# Autodesk Inventor assembly: Mark 4.5
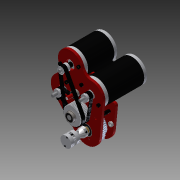
[picture p0: Inventor's stored thumbnail of the model, 180x180]
Saved by Autodesk Inventor 2013 (Build 170138000, 138)
## iProperties
Created: 2013-06-28
Part Number: Mark 4.5
Document SubType Name: Assembly
Designer: mvarma
Author: mvarma
## Documents named in this file (54)
- C:\Users\mvarma\Desktop\GRT 2013-2014 Gearbox\Mark 5\Mark 4.5.iam
- C:\Users\mvarma\Desktop\GRT 2013-2014 Gearbox\Mark 5\Plates\Mounting Plate.ipt
- C:\Users\mvarma\Desktop\GRT 2013-2014 Gearbox\Mark 5\Plates\Cim Plate.ipt
- C:\Users\mvarma\Desktop\GRT 2013-2014 Gearbox\Mark 5\Plates\Pnuematic Plate.ipt
- C:\Users\mvarma\Desktop\GRT 2013-2014 Gearbox\Mark 5\Plates\Main Connecting Standoff.ipt
- C:\Users\mvarma\Desktop\GRT 2013-2014 Gearbox\Mark 5\Pem Nuts\10-32 Clinch Style Pem Nut .091 Minimum Panel Thickness.ipt
- C:\Users\mvarma\Desktop\GRT 2013-2014 Gearbox\Mark 5\Pem Nuts\.25-20 Clinch Style Pem Nut .125 Minimum Panel Thickness.ipt
- C:\Users\mvarma\Desktop\GRT 2013-2014 Gearbox\Mark 5\Bearings\FR6-2ZZ - Hex.ipt
- C:\Users\mvarma\Desktop\GRT 2013-2014 Gearbox\Mark 5\Bearings\FR8-2RS.ipt
- C:\Users\mvarma\Desktop\GRT 2013-2014 Gearbox\Mark 5\Bearings\FR6-2RS.ipt
- C:\Users\mvarma\Desktop\GRT 2013-2014 Gearbox\Mark 5\Encoder\Encoder Mount.ipt
- C:\Users\mvarma\Desktop\GRT 2013-2014 Gearbox\Mark 5\Encoder\S4-120-250-N-S-B.ipt
- C:\Users\mvarma\Desktop\GRT 2013-2014 Gearbox\Mark 5\Shafts\Cluster Shaft.ipt
- C:\Users\mvarma\Desktop\GRT 2013-2014 Gearbox\Mark 5\Shafts\Flexible Shaft Coupler 6208K411.ipt
- C:\Users\mvarma\Desktop\GRT 2013-2014 Gearbox\Mark 5\Spacers\Cluster Shaft Spacer.ipt
- C:\Users\mvarma\Desktop\GRT 2013-2014 Gearbox\Mark 5\Gears\15T 20DP - .375 Hex Bore.ipt
- C:\Users\mvarma\Desktop\GRT 2013-2014 Gearbox\Mark 5\Gears\28T 20DP - .375 Hex Bore.ipt
- C:\Users\mvarma\Desktop\GRT 2013-2014 Gearbox\Mark 5\Shafts\Output Shaft.ipt
- C:\Users\mvarma\Desktop\GRT 2013-2014 Gearbox\Mark 5\Spacers\Shim 10 thou .500 Bore.ipt
- C:\Users\mvarma\Desktop\GRT 2013-2014 Gearbox\Mark 5\Bearings\R10-Open.ipt
- C:\Users\mvarma\Desktop\GRT 2013-2014 Gearbox\Mark 5\Gears\35T 20DP - .188 Ball Shifting Bore.ipt
- C:\Users\mvarma\Desktop\GRT 2013-2014 Gearbox\Mark 5\Gears\48T 20DP - .188 Ball Shifting Bore.ipt
- C:\Users\mvarma\Desktop\GRT 2013-2014 Gearbox\Mark 5\Bearings\Thrust Bearing Washer - .6250 Bore.ipt
- C:\Users\mvarma\Desktop\GRT 2013-2014 Gearbox\Mark 5\Spacers\Shim 10 thou .625 Bore.ipt
- C:\Users\mvarma\Desktop\GRT 2013-2014 Gearbox\Mark 5\Spacers\Shim 10 thou .375 Bore.ipt
- C:\Users\mvarma\Desktop\GRT 2013-2014 Gearbox\Mark 5\Pulleys\48T 3mm GT2 - .375 Hex Broach - Hubless.ipt
- C:\Users\mvarma\Desktop\GRT 2013-2014 Gearbox\Mark 5\Pem Nuts\4-40 Clinch Style Pem Nut .091 Minimum Panel Thickness.ipt
- C:\Users\mvarma\Desktop\GRT 2013-2014 Gearbox\Mark 5\Shafts\Tensioning Shaft.ipt
- C:\Users\mvarma\Desktop\GRT 2013-2014 Gearbox\Mark 5\Spacers\Belt Shaft Spacer 2.ipt
- C:\Users\mvarma\Desktop\GRT 2013-2014 Gearbox\Mark 5\Bearings\R4-2RS.ipt
- C:\Users\mvarma\Desktop\GRT 2013-2014 Gearbox\Mark 5\Motors\CIM Can.ipt
- C:\Users\mvarma\Desktop\GRT 2013-2014 Gearbox\Mark 5\Motors\Mini CIM Can.ipt
- C:\Users\mvarma\Desktop\GRT 2013-2014 Gearbox\Mark 5\Motors\Rotor.ipt
- C:\Users\mvarma\Desktop\GRT 2013-2014 Gearbox\Mark 5\Belts\267 mm Belt.ipt
- C:\Users\mvarma\Desktop\GRT 2013-2014 Gearbox\Mark 5\Belts\285 mm Belt.ipt
- C:\Users\mvarma\Desktop\GRT 2013-2014 Gearbox\Mark 5\Pulleys\16T 3mm GT2 - 8mm Key Broach.ipt
- C:\Users\mvarma\Desktop\GRT 2013-2014 Gearbox\Mark 5\Spacers\Cim Spacer.ipt
- C:\Users\mvarma\Desktop\GRT 2013-2014 Gearbox\Mark 5\Spacers\MiniCim Spacer.ipt
- C:\Users\mvarma\Desktop\GRT 2013-2014 Gearbox\Mark 5\Shafts\Ball Shifting Shaft.ipt
- C:\Users\mvarma\Desktop\GRT 2013-2014 Gearbox\Mark 5\Shafts\Output Shaft Insert.ipt
- C:\Users\mvarma\Desktop\GRT 2013-2014 Gearbox\Mark 5\Bearings\R3-2RS.ipt
- C:\Users\mvarma\Desktop\GRT 2013-2014 Gearbox\Mark 5\.0625 Spring Pin .2500 Long.ipt
- C:\Users\mvarma\Desktop\GRT 2013-2014 Gearbox\Mark 5\Pneumatic\Pneumatic Connector -Actuator Side.ipt
- C:\Users\mvarma\Desktop\GRT 2013-2014 Gearbox\Mark 5\Pneumatic\Pneumatic Connector -Shaft Side Cover.ipt
- C:\Users\mvarma\Desktop\GRT 2013-2014 Gearbox\Mark 5\Pneumatic\Pancake Pneumatic.iam
- C:\Users\mvarma\Desktop\GRT 2013-2014 Gearbox\Mark 5\Bolts\Button Head Cap Screw 4-40 Thread .125 Length.ipt
- C:\Users\mvarma\Desktop\GRT 2013-2014 Gearbox\Mark 5\Shafts\Output Shaft Hex Sleave.ipt
- C:\Users\mvarma\Desktop\GRT 2013-2014 Gearbox\Mark 5\Frame Segment.ipt
- C:\Users\mvarma\Desktop\GRT 2013-2014 Gearbox\Mark 5\Bolts\Socket Head Cap Screw 6-32 Thread 1.000 Length.ipt
- C:\Users\mvarma\Desktop\GRT 2013-2014 Gearbox\Mark 5\Plates\Cim Adjustment Block.ipt
- C:\Users\mvarma\Desktop\GRT 2013-2014 Gearbox\Mark 5\Bolts\Socket Head Cap Screw 6-32 Thread .500 Length.ipt
- C:\Users\mvarma\Desktop\GRT 2013-2014 Gearbox\Mark 5\Bolts\Socket Head Cap Screw 6-32 Thread .375 Length.ipt
- C:\Users\mvarma\Desktop\GRT 2013-2014 Gearbox\Mark 5\Bolts\Socket Head Cap Screw 10-32 Thread .750 Length.ipt
- C:\Users\mvarma\Desktop\GRT 2013-2014 Gearbox\Mark 5\Bolts\Socket Head Cap Screw 4-40 Thread 1.000 Length.ipt
## Components (85 placed, 53 different names)
1. Frame Segment:1 — Mate:228, Mate:229
2. Socket Head Cap Screw 4-40 Thread 1.000 Length:1 — Mate:270, Mate:272
3. Socket Head Cap Screw 4-40 Thread 1.000 Length:2 — Mate:271, Mate:273
4. 267 mm Belt:1 — Mate:174, Mate:175, Mate:179, Flush:2, Flush:3
5. 285 mm Belt:1 — Mate:176, Mate:177, Mate:178, Flush:1
6. Socket Head Cap Screw 6-32 Thread 1.000 Length:1 — Mate:232, Mate:234
7. Socket Head Cap Screw 6-32 Thread 1.000 Length:2 — Mate:231, Mate:233
8. S4-120-250-N-S-B:1 — Mate:66, Mate:67
9. Flexible Shaft Coupler 6208K411:1 — Mate:64, Mate:65, Mate:66, Mate:67
10. Encoder Mount:1 — Mate:225, Mate:226, Mate:227, Mate:231, Mate:232, Mate:233, Mate:234
11. Cim Spacer:1 — Mate:184, Mate:185
12. MiniCim Spacer:1 — Mate:187, Mate:188
13. Cim Spacer:2 — Mate:183, Mate:186
14. CIM Can:1 — Mate:153, Mate:154, Mate:155, Mate:163, Mate:166, Mate:185
15. CIM Can:2 — Mate:156, Mate:157, Mate:158, Mate:164, Mate:165, Mate:186
16. Mini CIM Can:1 — Mate:159, Mate:160, Mate:161, Mate:162, Mate:167, Mate:188, Mate:254
17. Rotor:1 — Mate:164, Mate:165, Mate:175, Mate:181, Mate:183
18. Rotor:2 — Mate:163, Mate:166, Mate:180, Mate:184
19. Rotor:3 — Mate:162, Mate:167, Mate:177, Mate:182, Mate:187
20. Pneumatic Connector -Actuator Side:1 — Mate:196, Mate:197, Mate:198, Mate:203, Mate:210, Mate:211
21. Pneumatic Connector -Shaft Side Cover:1 — Mate:196, Mate:197, Mate:198, Mate:201, Mate:214, Mate:219, Mate:220, Mate:221, Mate:222
22. Pancake Pneumatic:1 [sub-assembly] — Mate:209, Mate:210, Mate:211, Mate:212, Mate:213, Mate:270, Mate:271, Mate:272, Mate:273
23. Button Head Cap Screw 4-40 Thread .125 Length:1 — Mate:221, Mate:222
24. Button Head Cap Screw 4-40 Thread .125 Length:2 — Mate:219, Mate:220
25. 16T 3mm GT2 - 8mm Key Broach:1 — Mate:180, Flush:3
26. 16T 3mm GT2 - 8mm Key Broach:2 — Mate:181, Flush:2
27. 16T 3mm GT2 - 8mm Key Broach:3 — Mate:182, Flush:1
28. Main Connecting Standoff:3 — Mate:3, Mate:12, Mate:27, Mate:140
29. Main Connecting Standoff:5 — Mate:5, Mate:16, Mate:25
30. Main Connecting Standoff:8 — Mate:8, Mate:19, Mate:24
31. Socket Head Cap Screw 10-32 Thread .750 Length:1 — Mate:262, Mate:263
32. Socket Head Cap Screw 10-32 Thread .750 Length:2 — Mate:252, Mate:253
33. Socket Head Cap Screw 10-32 Thread .750 Length:3 — Mate:254, Mate:255
34. Socket Head Cap Screw 10-32 Thread .750 Length:4 — Mate:260, Mate:261
35. Socket Head Cap Screw 10-32 Thread .750 Length:5 — Mate:256, Mate:259
36. Socket Head Cap Screw 10-32 Thread .750 Length:6 — Mate:257, Mate:258
37. Mounting Plate:1 — Mate:3, Mate:5, Mate:8, Mate:24, Mate:25, Mate:27, Mate:31, Mate:34, Mate:36, Mate:40, Mate:42, Mate:45, Mate:48, Mate:49, Mate:50, Mate:51, Mate:53, Mate:55, Mate:56, Mate:57, Mate:68, Mate:73, Mate:74, Mate:225, Mate:226, Mate:227, Mate:229, Mate:235, Mate:236, Mate:237, Mate:243, Mate:244, Mate:245
38. FR8-2RS:1 — Mate:53, Mate:55, Mate:80, Mate:83
39. FR6-2RS:1 — Mate:56, Mate:57, Mate:72
40. Cim Plate:1 — Mate:12, Mate:16, Mate:19, Mate:58, Mate:59, Mate:60, Mate:61, Mate:114, Mate:115, Mate:139, Mate:140, Mate:141, Mate:142, Mate:153, Mate:154, Mate:155, Mate:156, Mate:157, Mate:158, Mate:159, Mate:160, Mate:161, Mate:174, Mate:176, Mate:252, Mate:253, Mate:255, Mate:256, Mate:257, Mate:258, Mate:259, Mate:260, Mate:261, Mate:262, Mate:263
41. FR6-2ZZ - Hex:1 — Mate:60, Mate:61, Mate:79, Mate:125
42. FR8-2RS:2 — Mate:58, Mate:59, Mate:214
43. Pnuematic Plate:1 — Mate:114, Mate:115, Mate:133, Mate:134, Mate:139, Mate:146, Mate:209, Mate:212, Mate:213, Mate:215, Mate:216, Mate:217, Mate:218
44. FR6-2RS:2 — Mate:133, Mate:134
45. Ball Shifting Shaft:1 — Mate:191, Mate:192, Mate:193, Mate:194, Mate:195, Mate:201
46. R3-2RS:1 — Mate:192, Mate:193, Mate:203
47. .0625 Spring Pin .2500 Long:1 — Mate:194, Mate:195
48. Cluster Shaft:1 — Mate:64, Mate:65, Mate:68, Mate:71, Mate:75, Mate:76, Mate:79, Mate:123, Mate:124, Mate:126, Mate:127, Mate:128, Mate:129
49. Cluster Shaft Spacer:1 — Mate:71, Mate:72, Mate:78
50. 15T 20DP - .375 Hex Bore:1 — Mate:74, Mate:76, Mate:77
51. 28T 20DP - .375 Hex Bore:1 — Mate:73, Mate:75, Mate:77, Mate:78
52. Shim 10 thou .375 Bore:1 — Mate:123, Mate:132
53. Shim 10 thou .500 Bore:2 — Mate:124, Mate:125, Mate:131
54. 48T 3mm GT2 - .375 Hex Broach - Hubless:1 — Mate:126, Mate:128, Mate:130, Mate:132, Mate:178
55. 48T 3mm GT2 - .375 Hex Broach - Hubless:2 — Mate:127, Mate:129, Mate:130, Mate:131, Mate:179
56. Output Shaft Insert:1 — Mate:189, Mate:190, Mate:191
57. Shim 10 thou .625 Bore:1 — Mate:96, Mate:97
58. Thrust Bearing Washer - .6250 Bore:2 — Mate:94, Mate:95, Mate:97
59. 48T 20DP - .188 Ball Shifting Bore:1 — Mate:92, Mate:93, Mate:95
60. R10-Open:1 — Mate:90, Mate:91, Mate:93
61. Thrust Bearing Washer - .6250 Bore:1 — Mate:88, Mate:89, Mate:91
62. 35T 20DP - .188 Ball Shifting Bore:1 — Mate:86, Mate:87, Mate:89
63. R10-Open:2 — Mate:84, Mate:85, Mate:87
64. Shim 10 thou .500 Bore:1 — Mate:81, Mate:82, Mate:83, Mate:85
65. Output Shaft:1 — Mate:80, Mate:81, Mate:82, Mate:84, Mate:86, Mate:88, Mate:90, Mate:92, Mate:94, Mate:96, Mate:189, Mate:190, Mate:223, Mate:224, Flush:4, Mate:228
66. Output Shaft Hex Sleave:1 — Mate:223, Mate:224, Flush:4
67. Tensioning Shaft:1 — Mate:141, Mate:142, Mate:143, Mate:149
68. Belt Shaft Spacer 2:1 — Mate:143, Mate:146, Mate:150
69. R4-2RS:1 — Mate:147, Mate:148, Mate:149, Mate:150
70. R4-2RS:2 — Mate:147, Mate:148
71. Cim Adjustment Block:1 — Mate:235, Mate:236, Mate:237, Mate:238, Mate:239, Mate:240, Mate:241, Mate:251
72. Cim Adjustment Block:2 — Mate:243, Mate:244, Mate:245, Mate:246, Mate:247, Mate:248, Mate:249, Mate:250
73. Socket Head Cap Screw 6-32 Thread .500 Length:1 — Mate:239, Mate:240
74. Socket Head Cap Screw 6-32 Thread .500 Length:2 — Mate:238, Mate:241
75. Socket Head Cap Screw 6-32 Thread .375 Length:2 — Mate:251
76. Socket Head Cap Screw 6-32 Thread .500 Length:4 — Mate:246, Mate:249
77. Socket Head Cap Screw 6-32 Thread .500 Length:5 — Mate:247, Mate:248
78. Socket Head Cap Screw 6-32 Thread .375 Length:1 — Mate:250
79. 10-32 Clinch Style Pem Nut .091 Minimum Panel Thickness:2 — Mate:34, Mate:40
80. 10-32 Clinch Style Pem Nut .091 Minimum Panel Thickness:4 — Mate:31, Mate:42
81. 10-32 Clinch Style Pem Nut .091 Minimum Panel Thickness:8 — Mate:36, Mate:45
82. .25-20 Clinch Style Pem Nut .125 Minimum Panel Thickness:1 — Mate:49, Mate:50
83. .25-20 Clinch Style Pem Nut .125 Minimum Panel Thickness:2 — Mate:48, Mate:51
84. 4-40 Clinch Style Pem Nut .091 Minimum Panel Thickness:1 — Mate:216, Mate:218
85. 4-40 Clinch Style Pem Nut .091 Minimum Panel Thickness:2 — Mate:215, Mate:217
## Relationships (188: Mate 182, Flush 4, Tangent 2)
- Mate:3: Main Connecting Standoff:3 ↔ Mounting Plate:1
- Mate:5: Main Connecting Standoff:5 ↔ Mounting Plate:1
- Mate:8: Main Connecting Standoff:8 ↔ Mounting Plate:1
- Mate:12: Main Connecting Standoff:3 ↔ Cim Plate:1
- Mate:16: Main Connecting Standoff:5 ↔ Cim Plate:1
- Mate:19: Main Connecting Standoff:8 ↔ Cim Plate:1
- Mate:24: Main Connecting Standoff:8 ↔ Mounting Plate:1
- Mate:25: Main Connecting Standoff:5 ↔ Mounting Plate:1
- Mate:27: Main Connecting Standoff:3 ↔ Mounting Plate:1
- Mate:31: Mounting Plate:1 ↔ 10-32 Clinch Style Pem Nut .091 Minimum Panel Thickness:4
- Mate:34: Mounting Plate:1 ↔ 10-32 Clinch Style Pem Nut .091 Minimum Panel Thickness:2
- Mate:36: Mounting Plate:1 ↔ 10-32 Clinch Style Pem Nut .091 Minimum Panel Thickness:8
- Mate:40: Mounting Plate:1 ↔ 10-32 Clinch Style Pem Nut .091 Minimum Panel Thickness:2
- Mate:42: Mounting Plate:1 ↔ 10-32 Clinch Style Pem Nut .091 Minimum Panel Thickness:4
- Mate:45: Mounting Plate:1 ↔ 10-32 Clinch Style Pem Nut .091 Minimum Panel Thickness:8
- Mate:48: Mounting Plate:1 ↔ .25-20 Clinch Style Pem Nut .125 Minimum Panel Thickness:2
- Mate:49: Mounting Plate:1 ↔ .25-20 Clinch Style Pem Nut .125 Minimum Panel Thickness:1
- Mate:50: Mounting Plate:1 ↔ .25-20 Clinch Style Pem Nut .125 Minimum Panel Thickness:1
- Mate:51: Mounting Plate:1 ↔ .25-20 Clinch Style Pem Nut .125 Minimum Panel Thickness:2
- Mate:53: Mounting Plate:1 ↔ FR8-2RS:1
- Mate:55: Mounting Plate:1 ↔ FR8-2RS:1
- Mate:56: Mounting Plate:1 ↔ FR6-2RS:1
- Mate:57: Mounting Plate:1 ↔ FR6-2RS:1
- Mate:58: Cim Plate:1 ↔ FR8-2RS:2
- Mate:59: Cim Plate:1 ↔ FR8-2RS:2
- Mate:60: Cim Plate:1 ↔ FR6-2ZZ - Hex:1
- Mate:61: Cim Plate:1 ↔ FR6-2ZZ - Hex:1
- Mate:64: Flexible Shaft Coupler 6208K411:1 ↔ Cluster Shaft:1
- Mate:65: Flexible Shaft Coupler 6208K411:1 ↔ Cluster Shaft:1
- Mate:66: S4-120-250-N-S-B:1 ↔ Flexible Shaft Coupler 6208K411:1
- Mate:67: S4-120-250-N-S-B:1 ↔ Flexible Shaft Coupler 6208K411:1
- Mate:68: Mounting Plate:1 ↔ Cluster Shaft:1
- Mate:71: Cluster Shaft:1 ↔ Cluster Shaft Spacer:1
- Mate:72: FR6-2RS:1 ↔ Cluster Shaft Spacer:1
- Mate:73: Mounting Plate:1 ↔ 28T 20DP - .375 Hex Bore:1
- Mate:74: Mounting Plate:1 ↔ 15T 20DP - .375 Hex Bore:1
- Mate:75: Cluster Shaft:1 ↔ 28T 20DP - .375 Hex Bore:1
- Mate:76: Cluster Shaft:1 ↔ 15T 20DP - .375 Hex Bore:1
- Mate:77: 15T 20DP - .375 Hex Bore:1 ↔ 28T 20DP - .375 Hex Bore:1
- Mate:78: Cluster Shaft Spacer:1 ↔ 28T 20DP - .375 Hex Bore:1
- Mate:79: FR6-2ZZ - Hex:1 ↔ Cluster Shaft:1
- Mate:80: FR8-2RS:1 ↔ Output Shaft:1
- Mate:81: Shim 10 thou .500 Bore:1 ↔ Output Shaft:1
- Mate:82: Shim 10 thou .500 Bore:1 ↔ Output Shaft:1
- Mate:83: FR8-2RS:1 ↔ Shim 10 thou .500 Bore:1
- Mate:84: R10-Open:2 ↔ Output Shaft:1
- Mate:85: R10-Open:2 ↔ Shim 10 thou .500 Bore:1
- Mate:86: 35T 20DP - .188 Ball Shifting Bore:1 ↔ Output Shaft:1
- Mate:87: 35T 20DP - .188 Ball Shifting Bore:1 ↔ R10-Open:2
- Mate:88: Thrust Bearing Washer - .6250 Bore:1 ↔ Output Shaft:1
- Mate:89: Thrust Bearing Washer - .6250 Bore:1 ↔ 35T 20DP - .188 Ball Shifting Bore:1
- Mate:90: R10-Open:1 ↔ Output Shaft:1
- Mate:91: R10-Open:1 ↔ Thrust Bearing Washer - .6250 Bore:1
- Mate:92: 48T 20DP - .188 Ball Shifting Bore:1 ↔ Output Shaft:1
- Mate:93: 48T 20DP - .188 Ball Shifting Bore:1 ↔ R10-Open:1
- Mate:94: Thrust Bearing Washer - .6250 Bore:2 ↔ Output Shaft:1
- Mate:95: Thrust Bearing Washer - .6250 Bore:2 ↔ 48T 20DP - .188 Ball Shifting Bore:1
- Mate:96: Shim 10 thou .625 Bore:1 ↔ Output Shaft:1
- Mate:97: Shim 10 thou .625 Bore:1 ↔ Thrust Bearing Washer - .6250 Bore:2
- Mate:114: Cim Plate:1 ↔ Pnuematic Plate:1
- Mate:115: Cim Plate:1 ↔ Pnuematic Plate:1
- Mate:123: Cluster Shaft:1 ↔ Shim 10 thou .375 Bore:1
- Mate:124: Cluster Shaft:1 ↔ Shim 10 thou .500 Bore:2
- Mate:125: FR6-2ZZ - Hex:1 ↔ Shim 10 thou .500 Bore:2
- Mate:126: Cluster Shaft:1 ↔ 48T 3mm GT2 - .375 Hex Broach - Hubless:1
- Mate:127: Cluster Shaft:1 ↔ 48T 3mm GT2 - .375 Hex Broach - Hubless:2
- Mate:128: Cluster Shaft:1 ↔ 48T 3mm GT2 - .375 Hex Broach - Hubless:1
- Mate:129: Cluster Shaft:1 ↔ 48T 3mm GT2 - .375 Hex Broach - Hubless:2
- Mate:130: 48T 3mm GT2 - .375 Hex Broach - Hubless:1 ↔ 48T 3mm GT2 - .375 Hex Broach - Hubless:2
- Mate:131: Shim 10 thou .500 Bore:2 ↔ 48T 3mm GT2 - .375 Hex Broach - Hubless:2
- Mate:132: Shim 10 thou .375 Bore:1 ↔ 48T 3mm GT2 - .375 Hex Broach - Hubless:1
- Mate:133: Pnuematic Plate:1 ↔ FR6-2RS:2
- Mate:134: Pnuematic Plate:1 ↔ FR6-2RS:2
- Mate:139: Cim Plate:1 ↔ Pnuematic Plate:1
- Mate:140: Main Connecting Standoff:3 ↔ Cim Plate:1
- Mate:141: Cim Plate:1 ↔ Tensioning Shaft:1
- Mate:142: Cim Plate:1 ↔ Tensioning Shaft:1
- Mate:143: Tensioning Shaft:1 ↔ Belt Shaft Spacer 2:1
- Mate:146: Pnuematic Plate:1 ↔ Belt Shaft Spacer 2:1
- Mate:147: R4-2RS:1 ↔ R4-2RS:2
- Mate:148: R4-2RS:1 ↔ R4-2RS:2
- Mate:149: Tensioning Shaft:1 ↔ R4-2RS:1
- Mate:150: Belt Shaft Spacer 2:1 ↔ R4-2RS:1
- Mate:153: CIM Can:1 ↔ Cim Plate:1
- Mate:154: CIM Can:1 ↔ Cim Plate:1
- Mate:155: CIM Can:1 ↔ Cim Plate:1
- Mate:156: CIM Can:2 ↔ Cim Plate:1
- Mate:157: CIM Can:2 ↔ Cim Plate:1
- Mate:158: CIM Can:2 ↔ Cim Plate:1
- Mate:159: Mini CIM Can:1 ↔ Cim Plate:1
- Mate:160: Mini CIM Can:1 ↔ Cim Plate:1
- Mate:161: Mini CIM Can:1 ↔ Cim Plate:1
- Mate:162: Mini CIM Can:1 ↔ Rotor:3
- Mate:163: CIM Can:1 ↔ Rotor:2
- Mate:164: CIM Can:2 ↔ Rotor:1
- Mate:165: CIM Can:2 ↔ Rotor:1
- Mate:166: CIM Can:1 ↔ Rotor:2
- Mate:167: Mini CIM Can:1 ↔ Rotor:3
- Mate:174: 267 mm Belt:1 ↔ Cim Plate:1
- Mate:175: 267 mm Belt:1 ↔ Rotor:1
- Mate:176: 285 mm Belt:1 ↔ Cim Plate:1
- Mate:177: 285 mm Belt:1 ↔ Rotor:3
- Mate:178: 285 mm Belt:1 ↔ 48T 3mm GT2 - .375 Hex Broach - Hubless:1
- Mate:179: 267 mm Belt:1 ↔ 48T 3mm GT2 - .375 Hex Broach - Hubless:2
- Mate:180: Rotor:2 ↔ 16T 3mm GT2 - 8mm Key Broach:1
- Mate:181: Rotor:1 ↔ 16T 3mm GT2 - 8mm Key Broach:2
- Mate:182: Rotor:3 ↔ 16T 3mm GT2 - 8mm Key Broach:3
- Flush:1: 285 mm Belt:1 ↔ 16T 3mm GT2 - 8mm Key Broach:3
- Flush:2: 267 mm Belt:1 ↔ 16T 3mm GT2 - 8mm Key Broach:2
- Flush:3: 267 mm Belt:1 ↔ 16T 3mm GT2 - 8mm Key Broach:1
- Mate:183: Cim Spacer:2 ↔ Rotor:1
- Mate:184: Cim Spacer:1 ↔ Rotor:2
- Mate:185: Cim Spacer:1 ↔ CIM Can:1
- Mate:186: Cim Spacer:2 ↔ CIM Can:2
- Mate:187: MiniCim Spacer:1 ↔ Rotor:3
- Mate:188: MiniCim Spacer:1 ↔ Mini CIM Can:1
- Mate:189: Output Shaft Insert:1 ↔ Output Shaft:1
- Mate:190: Output Shaft Insert:1 ↔ Output Shaft:1
- Mate:191: Ball Shifting Shaft:1 ↔ Output Shaft Insert:1
- Mate:192: Ball Shifting Shaft:1 ↔ R3-2RS:1
- Mate:193: Ball Shifting Shaft:1 ↔ R3-2RS:1
- Mate:194: Ball Shifting Shaft:1 ↔ .0625 Spring Pin .2500 Long:1
- Mate:195: Ball Shifting Shaft:1 ↔ .0625 Spring Pin .2500 Long:1
- Mate:196: Pneumatic Connector -Actuator Side:1 ↔ Pneumatic Connector -Shaft Side Cover:1
- Mate:197: Pneumatic Connector -Actuator Side:1 ↔ Pneumatic Connector -Shaft Side Cover:1
- Mate:198: Pneumatic Connector -Actuator Side:1 ↔ Pneumatic Connector -Shaft Side Cover:1
- Mate:201: Pneumatic Connector -Shaft Side Cover:1 ↔ Ball Shifting Shaft:1
- Mate:203: Pneumatic Connector -Actuator Side:1 ↔ R3-2RS:1
- Mate:209: Pancake Pneumatic:1 ↔ Pnuematic Plate:1
- Mate:210: Pneumatic Connector -Actuator Side:1 ↔ Pancake Pneumatic:1
- Mate:211: Pneumatic Connector -Actuator Side:1 ↔ Pancake Pneumatic:1
- Mate:212: Pancake Pneumatic:1 ↔ Pnuematic Plate:1
- Mate:213: Pancake Pneumatic:1 ↔ Pnuematic Plate:1
- Mate:214 (8.8582 mm): Pneumatic Connector -Shaft Side Cover:1 ↔ FR8-2RS:2
- Mate:215: Pnuematic Plate:1 ↔ 4-40 Clinch Style Pem Nut .091 Minimum Panel Thickness:2
- Mate:216: Pnuematic Plate:1 ↔ 4-40 Clinch Style Pem Nut .091 Minimum Panel Thickness:1
- Mate:217: Pnuematic Plate:1 ↔ 4-40 Clinch Style Pem Nut .091 Minimum Panel Thickness:2
- Mate:218: Pnuematic Plate:1 ↔ 4-40 Clinch Style Pem Nut .091 Minimum Panel Thickness:1
- Mate:219: Pneumatic Connector -Shaft Side Cover:1 ↔ Button Head Cap Screw 4-40 Thread .125 Length:2
- Mate:220: Pneumatic Connector -Shaft Side Cover:1 ↔ Button Head Cap Screw 4-40 Thread .125 Length:2
- Mate:221: Pneumatic Connector -Shaft Side Cover:1 ↔ Button Head Cap Screw 4-40 Thread .125 Length:1
- Mate:222: Pneumatic Connector -Shaft Side Cover:1 ↔ Button Head Cap Screw 4-40 Thread .125 Length:1
- Mate:223: Output Shaft:1 ↔ Output Shaft Hex Sleave:1
- Mate:224: Output Shaft:1 ↔ Output Shaft Hex Sleave:1
- Flush:4: Output Shaft:1 ↔ Output Shaft Hex Sleave:1
- Mate:225: Encoder Mount:1 ↔ Mounting Plate:1
- Mate:226: Encoder Mount:1 ↔ Mounting Plate:1
- Mate:227: Encoder Mount:1 ↔ Mounting Plate:1
- Mate:228: Frame Segment:1 ↔ Output Shaft:1
- Mate:229: Frame Segment:1 ↔ Mounting Plate:1
- Mate:231: Socket Head Cap Screw 6-32 Thread 1.000 Length:2 ↔ Encoder Mount:1
- Mate:232: Socket Head Cap Screw 6-32 Thread 1.000 Length:1 ↔ Encoder Mount:1
- Mate:233: Socket Head Cap Screw 6-32 Thread 1.000 Length:2 ↔ Encoder Mount:1
- Mate:234: Socket Head Cap Screw 6-32 Thread 1.000 Length:1 ↔ Encoder Mount:1
- Mate:235: Mounting Plate:1 ↔ Cim Adjustment Block:1
- Mate:236: Mounting Plate:1 ↔ Cim Adjustment Block:1
- Mate:237: Mounting Plate:1 ↔ Cim Adjustment Block:1
- Mate:238: Cim Adjustment Block:1 ↔ Socket Head Cap Screw 6-32 Thread .500 Length:2
- Mate:239: Cim Adjustment Block:1 ↔ Socket Head Cap Screw 6-32 Thread .500 Length:1
- Mate:240: Cim Adjustment Block:1 ↔ Socket Head Cap Screw 6-32 Thread .500 Length:1
- Mate:241: Cim Adjustment Block:1 ↔ Socket Head Cap Screw 6-32 Thread .500 Length:2
- [Tangent]: CIM Can:2 ↔ Socket Head Cap Screw 6-32 Thread .375 Length:2
- Mate:243: Mounting Plate:1 ↔ Cim Adjustment Block:2
- Mate:244: Mounting Plate:1 ↔ Cim Adjustment Block:2
- Mate:245: Mounting Plate:1 ↔ Cim Adjustment Block:2
- Mate:246: Cim Adjustment Block:2 ↔ Socket Head Cap Screw 6-32 Thread .500 Length:4
- Mate:247: Cim Adjustment Block:2 ↔ Socket Head Cap Screw 6-32 Thread .500 Length:5
- Mate:248: Cim Adjustment Block:2 ↔ Socket Head Cap Screw 6-32 Thread .500 Length:5
- Mate:249: Cim Adjustment Block:2 ↔ Socket Head Cap Screw 6-32 Thread .500 Length:4
- [Tangent]: Mini CIM Can:1 ↔ Socket Head Cap Screw 6-32 Thread .375 Length:1
- Mate:250: Cim Adjustment Block:2 ↔ Socket Head Cap Screw 6-32 Thread .375 Length:1
- Mate:251: Cim Adjustment Block:1 ↔ Socket Head Cap Screw 6-32 Thread .375 Length:2
- Mate:252: Socket Head Cap Screw 10-32 Thread .750 Length:2 ↔ Cim Plate:1
- Mate:253: Socket Head Cap Screw 10-32 Thread .750 Length:2 ↔ Cim Plate:1
- Mate:254: Mini CIM Can:1 ↔ Socket Head Cap Screw 10-32 Thread .750 Length:3
- Mate:255: Socket Head Cap Screw 10-32 Thread .750 Length:3 ↔ Cim Plate:1
- Mate:256: Socket Head Cap Screw 10-32 Thread .750 Length:5 ↔ Cim Plate:1
- Mate:257: Socket Head Cap Screw 10-32 Thread .750 Length:6 ↔ Cim Plate:1
- Mate:258: Socket Head Cap Screw 10-32 Thread .750 Length:6 ↔ Cim Plate:1
- Mate:259: Socket Head Cap Screw 10-32 Thread .750 Length:5 ↔ Cim Plate:1
- Mate:260: Socket Head Cap Screw 10-32 Thread .750 Length:4 ↔ Cim Plate:1
- Mate:261: Socket Head Cap Screw 10-32 Thread .750 Length:4 ↔ Cim Plate:1
- Mate:262: Socket Head Cap Screw 10-32 Thread .750 Length:1 ↔ Cim Plate:1
- Mate:263: Socket Head Cap Screw 10-32 Thread .750 Length:1 ↔ Cim Plate:1
- Mate:270: Socket Head Cap Screw 4-40 Thread 1.000 Length:1 ↔ Pancake Pneumatic:1
- Mate:271: Socket Head Cap Screw 4-40 Thread 1.000 Length:2 ↔ Pancake Pneumatic:1
- Mate:272: Socket Head Cap Screw 4-40 Thread 1.000 Length:1 ↔ Pancake Pneumatic:1
- Mate:273: Socket Head Cap Screw 4-40 Thread 1.000 Length:2 ↔ Pancake Pneumatic:1
